# Autodesk Inventor assembly: zlozenie_blotnik_v3
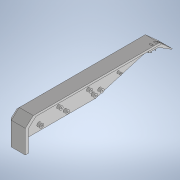
[picture p0: Inventor's stored thumbnail of the model, 180x180]
Saved by Autodesk Inventor 2022.3 (Build 263350000, 350)
## iProperties
Created: 2022-10-27
Part Number: zlozenie_blotnik_v3
Document SubType Name: Assembly
Designer: komputer
Author: komputer
## Documents named in this file (6)
- C:\Users\komputer\Desktop\zlozenie_blotnik_v3.iam
- C:\Users\komputer\Desktop\błotnik_v2.ipt
- C:\Users\komputer\zaślepka-1.ipt
- C:\Users\komputer\zaslepka_sruby-1.ipt
- C:\Users\komputer\Desktop\zaslepka_sruby-1.ipt
- C:\Users\komputer\Documents\Inventor\Content Center Files\R2022\en-US\U 2494(1)\Unbrako - M4 x  30(6).ipt
## Components (6 placed, 4 different names)
1. błotnik_v2:1 — Flush:1, Flush:2, Flush:3, Flush:4, Flush:5, Mate:1, Flush:6, Mate:2, Mate:5
2. zaślepka-1:1 — Flush:1, Flush:2, Flush:3, Mate:3, Mate:4
3. zaslepka_sruby-1:1 — Flush:4, Flush:5
4. zaslepka_sruby-1:2 — Mate:1, Flush:6
5. Unbrako Hex Socket Cap - Metric M4 x 30:1 — Mate:2, Mate:3
6. Unbrako Hex Socket Cap - Metric M4 x 30:2 — Mate:4, Mate:5
## Relationships (11: Flush 6, Mate 5)
- Flush:1: błotnik_v2:1 ↔ zaślepka-1:1
- Flush:2: błotnik_v2:1 ↔ zaślepka-1:1
- Flush:3: błotnik_v2:1 ↔ zaślepka-1:1
- Flush:4: błotnik_v2:1 ↔ zaslepka_sruby-1:1
- Flush:5: błotnik_v2:1 ↔ zaslepka_sruby-1:1
- Mate:1: błotnik_v2:1 ↔ zaslepka_sruby-1:2
- Flush:6: błotnik_v2:1 ↔ zaslepka_sruby-1:2
- Mate:2: błotnik_v2:1 ↔ Unbrako Hex Socket Cap - Metric M4 x 30:1
- Mate:3: zaślepka-1:1 ↔ Unbrako Hex Socket Cap - Metric M4 x 30:1
- Mate:4: zaślepka-1:1 ↔ Unbrako Hex Socket Cap - Metric M4 x 30:2
- Mate:5: błotnik_v2:1 ↔ Unbrako Hex Socket Cap - Metric M4 x 30:2
